# Autodesk Inventor assembly: Intel RealSense T265
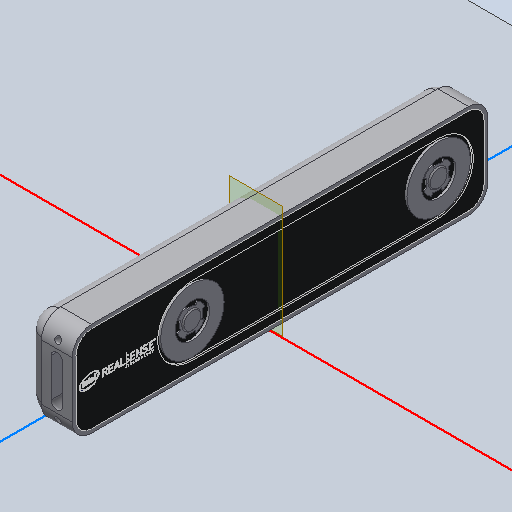
[picture p0: Inventor's stored thumbnail of the model, 512x512]
Saved by Autodesk Inventor 2022 (Build 260153000, 153)
## iProperties
Created: 2020-09-15
Part Number: Intel RealSense T265
Material: Типовые
Document SubType Name: Assembly
Designer: Петров Иван
Mass: 224.829 g
Surface Area: 142.298 cm^2
Volume: 28.6406 cm^3
Density: 7.85 g/cm^3
Sending System: Autodesk Translation Framework v9.3.0.1241
Preprocessor: ST-DEVELOPER v18.1
Title: C:/Users/Pranshu Tople/Downloads/Intel_RealSense_Tracking_Camera_T265.stp_/Intel RealSense T265.step
## Documents named in this file (3)
- D:\IVAN\Ivan_desktop\Kvantorium\Projects\YouBotRobot\design\standart_components\Realsense\D200\Intel RealSense T265.iam
- D:\IVAN\Ivan_desktop\Kvantorium\Projects\YouBotRobot\design\standart_components\Realsense\D200\body.ipt
- D:\IVAN\Ivan_desktop\Kvantorium\Projects\YouBotRobot\design\standart_components\Realsense\D200\cover.ipt
## Components (2 placed, 2 different names)
1. body:1 — Совмещение:1, Угол:1
2. cover:1
## Relationships (2: Mate 1, Angle 1)
- Совмещение:1 [Mate]: body:1
- Угол:1 [Angle] (0 deg): body:1
